# Autodesk Inventor assembly: 6P 8T Sprocket, No Insert_MIR
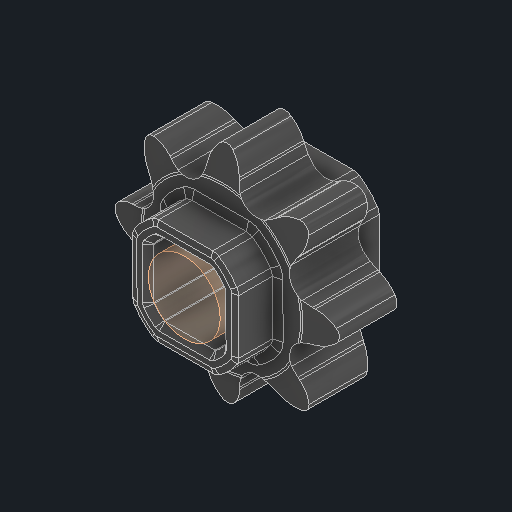
[picture p0: Inventor's stored thumbnail of the model, 512x512]
Saved by Autodesk Inventor 2024 (Build 280153000, 153)
## iProperties
Created: 2022-08-02
Part Number: 6P 8T Sprocket, No Insert_MIR
Document SubType Name: Assembly
Designer: Averey Ku
Author: ylu12
## Documents named in this file (2)
- D:\vex_robotics\hardware\cad\spades_v0.1\intake\mirrored_parts\6P 8T Sprocket, No Insert_MIR.iam
- D:\vex_robotics\hardware\cad\spades_v0.1\intake\mirrored_parts\6P 8T Sprocket_MIR.ipt
## Components (1 placed, 1 different names)
1. 6P 8T Sprocket_MIR:1 — Flush:3, Mate:6, Mate:5
## Relationships (3: Mate 2, Flush 1)
- Flush:3: 6P 8T Sprocket_MIR:1
- Mate:6: 6P 8T Sprocket_MIR:1
- Mate:5: 6P 8T Sprocket_MIR:1
